# Autodesk Inventor assembly: PK_Arm_V1
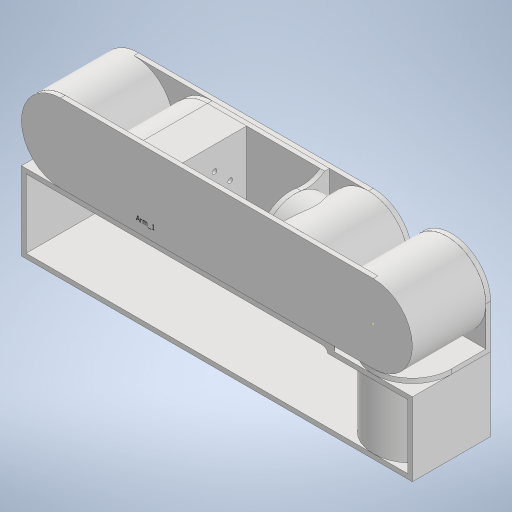
[picture p0: Inventor's stored thumbnail of the model, 512x512]
Saved by Autodesk Inventor 2023 (Build 270158000, 158)
## iProperties
Created: 2022-04-08
Part Number: PK_Arm_V1
Document SubType Name: Assembly
Designer: device
Author: device
## Documents named in this file (8)
- D:\NTNU\PK_Arm_V1.iam
- D:\NTNU\Arm_1.ipt
- D:\NTNU\Arm_2.ipt
- D:\NTNU\Arm_3.ipt
- D:\NTNU\Arm_4.ipt
- D:\NTNU\Arm_5.ipt
- D:\NTNU\Base_1.ipt
- D:\NTNU\Base_box.ipt
## Components (7 placed, 7 different names)
1. Base_box:1 — 齊平:1, 齊平:2, 齊平:3, 貼合:13, 貼合:14, 角度:0
2. Base_1:1 — 貼合:11, 貼合:12, 貼合:13, 貼合:14, 角度:0, 角度:1
3. Arm_1:1 — 貼合:1, 貼合:2, 貼合:11, 貼合:12, 角度:1, 角度:2
4. Arm_2:1 — 貼合:1, 貼合:2, 貼合:3, 貼合:4, 角度:2, 角度:3
5. Arm_3:1 — 貼合:3, 貼合:4, 貼合:7, 貼合:8, 角度:3, 角度:4
6. Arm_4:1 — 貼合:7, 貼合:8, 貼合:9, 貼合:10, 角度:4, 角度:5
7. Arm_5:1 — 貼合:9, 貼合:10, 角度:5
## Relationships (21: Mate 12, Angle 6, Flush 3)
- 齊平:1 [Flush]: Base_box:1
- 齊平:2 [Flush]: Base_box:1
- 齊平:3 [Flush]: Base_box:1
- 貼合:1 [Mate]: Arm_1:1 ↔ Arm_2:1
- 貼合:2 [Mate]: Arm_1:1 ↔ Arm_2:1
- 貼合:3 [Mate]: Arm_2:1 ↔ Arm_3:1
- 貼合:4 [Mate]: Arm_2:1 ↔ Arm_3:1
- 貼合:7 [Mate]: Arm_3:1 ↔ Arm_4:1
- 貼合:8 [Mate]: Arm_3:1 ↔ Arm_4:1
- 貼合:9 [Mate]: Arm_4:1 ↔ Arm_5:1
- 貼合:10 [Mate]: Arm_4:1 ↔ Arm_5:1
- 貼合:11 [Mate]: Base_1:1 ↔ Arm_1:1
- 貼合:12 [Mate]: Base_1:1 ↔ Arm_1:1
- 貼合:13 [Mate]: Base_box:1 ↔ Base_1:1
- 貼合:14 [Mate]: Base_box:1 ↔ Base_1:1
- 角度:0 [Angle] (0 deg): Base_box:1 ↔ Base_1:1
- 角度:1 [Angle] (0 deg): Base_1:1 ↔ Arm_1:1
- 角度:2 [Angle] (0 deg): Arm_1:1 ↔ Arm_2:1
- 角度:3 [Angle] (0 deg): Arm_2:1 ↔ Arm_3:1
- 角度:4 [Angle] (0 deg): Arm_3:1 ↔ Arm_4:1
- 角度:5 [Angle] (0 deg): Arm_4:1 ↔ Arm_5:1
